# Autodesk Inventor assembly: lcd
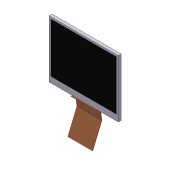
[picture p0: Inventor's stored thumbnail of the model, 180x180]
Saved by Autodesk Inventor 2014 (Build 180170000, 170)
## iProperties
Created: 2013-06-20
Part Number: lcd
Document SubType Name: Assembly
Designer: Administrator
Author: Administrator
## Documents named in this file (4)
- C:\Users\user\Desktop\beagleboy\lcd.iam
- C:\Users\user\Desktop\beagleboy\lcd_frame.ipt
- C:\Users\user\Desktop\beagleboy\lcd_glass.ipt
- C:\Users\user\Desktop\beagleboy\lcd_ribbon.ipt
## Components (3 placed, 3 different names)
1. lcd_frame:1 — Mate:1, Mate:2, Mate:3, Flush:1, Mate:4, Mate:5
2. lcd_glass:1 — Mate:1, Mate:2, Mate:3
3. lcd_ribbon:1 — Flush:1, Mate:4, Mate:5
## Relationships (6: Mate 5, Flush 1)
- Mate:1: lcd_frame:1 ↔ lcd_glass:1
- Mate:2: lcd_frame:1 ↔ lcd_glass:1
- Mate:3: lcd_frame:1 ↔ lcd_glass:1
- Flush:1 (15.7 mm): lcd_frame:1 ↔ lcd_ribbon:1
- Mate:4: lcd_frame:1 ↔ lcd_ribbon:1
- Mate:5 (-0.508 mm): lcd_frame:1 ↔ lcd_ribbon:1
